# Autodesk Inventor assembly: Assembly1
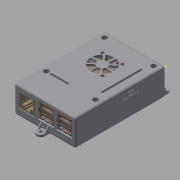
[picture p0: Inventor's stored thumbnail of the model, 180x180]
Saved by Autodesk Inventor 2017 (Build 210142000, 142)
## iProperties
Created: 2016-12-17
Part Number: Assembly1
Document SubType Name: Assembly
Designer: bartv
Author: bartv
## Documents named in this file (6)
- D:\bartv\Documents\Inventor\RPI3_Case\Assembly1.iam
- D:\bartv\Documents\Inventor\RPI3_Case\Bodem.ipt
- D:\bartv\Documents\Inventor\RPI3_Case\RPi3_ModelB.iam
- D:\bartv\Documents\Inventor\RPI3_Case\Deksel.ipt
- D:\bartv\Documents\Inventor\RPI3_Case\tactileswitch-short.ipt
- D:\bartv\Documents\Inventor\RPI3_Case\Klepje.ipt
## Components (5 placed, 5 different names)
1. Bodem:1 — Mate:1, Mate:2, Mate:3, Mate:6
2. RPi3_ModelB:1 [sub-assembly] — Mate:1, Mate:2, Mate:3, Mate:4, Mate:5
3. Deksel:1 — Mate:4, Mate:5, Mate:6, Mate:7, Mate:8, Mate:9, Mate:10, Mate:11, Mate:12
4. tactileswitch-short:1 — Mate:7, Mate:8, Mate:9
5. Klepje:1 — Mate:10, Mate:11, Mate:12
## Relationships (12: Mate 12)
- Mate:1: Bodem:1 ↔ RPi3_ModelB:1
- Mate:2: Bodem:1 ↔ RPi3_ModelB:1
- Mate:3: Bodem:1 ↔ RPi3_ModelB:1
- Mate:4: RPi3_ModelB:1 ↔ Deksel:1
- Mate:5: RPi3_ModelB:1 ↔ Deksel:1
- Mate:6: Bodem:1 ↔ Deksel:1
- Mate:7: Deksel:1 ↔ tactileswitch-short:1
- Mate:8: Deksel:1 ↔ tactileswitch-short:1
- Mate:9: Deksel:1 ↔ tactileswitch-short:1
- Mate:10: Deksel:1 ↔ Klepje:1
- Mate:11: Deksel:1 ↔ Klepje:1
- Mate:12: Deksel:1 ↔ Klepje:1
